# Autodesk Inventor assembly: Granny Gearbox Output Plate Routing Template (8-sheet)
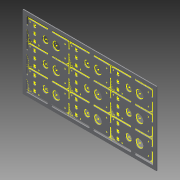
[picture p0: Inventor's stored thumbnail of the model, 180x180]
Saved by Autodesk Inventor 2015 (Build 190159000, 159)
## iProperties
Created: 2016-02-25
Part Number: Granny Gearbox Output Plate Routing Template (8-sheet)
Document SubType Name: Assembly
Designer: sethbattis
Author: sethbattis
## Documents named in this file (4)
- \\area51\team3566\cad\FRC 2016\Granny Gearbox Output Plate Routing Template (8-sheet).iam
- \\area51\team3566\cad\FRC 2016\Granny Gearbox Output Plate Routing Template (border tabs).ipt
- \\area51\team3566\cad\FRC 2016\Granny Gearbox Routing Template Horizontal Tabs.ipt
- \\area51\team3566\cad\FRC 2016\Granny Gearbox Routing Template Vertical Tabs.ipt
## Components (21 placed, 3 different names)
1. Granny Gearbox Output Plate Routing Template (border tabs):1 — Rigid:3, Rigid:4, Rigid:14, Rigid:18
2. Granny Gearbox Output Plate Routing Template (border tabs):2 — Rigid:1, Rigid:2, Rigid:3, Rigid:13
3. Granny Gearbox Output Plate Routing Template (border tabs):3 — Rigid:2, Rigid:7
4. Granny Gearbox Output Plate Routing Template (border tabs):4 — Rigid:6, Rigid:8, Rigid:10
5. Granny Gearbox Output Plate Routing Template (border tabs):5 — Rigid:5, Rigid:6, Rigid:11, Rigid:20
6. Granny Gearbox Output Plate Routing Template (border tabs):6 — Rigid:4, Rigid:5, Rigid:19
7. Granny Gearbox Output Plate Routing Template (border tabs):7 — Rigid:8, Rigid:9, Rigid:17
8. Granny Gearbox Output Plate Routing Template (border tabs):8 — Rigid:7, Rigid:16
9. Granny Gearbox Output Plate Routing Template (border tabs):9 — Rigid:1, Rigid:12, Rigid:15
10. Granny Gearbox Routing Template Horizontal Tabs:1 — Rigid:9
11. Granny Gearbox Routing Template Horizontal Tabs:2 — Rigid:10
12. Granny Gearbox Routing Template Horizontal Tabs:3 — Rigid:11
13. Granny Gearbox Routing Template Horizontal Tabs:4 — Rigid:12
14. Granny Gearbox Routing Template Horizontal Tabs:5 — Rigid:13
15. Granny Gearbox Routing Template Horizontal Tabs:6 — Rigid:14
16. Granny Gearbox Routing Template Vertical Tabs:1 — Rigid:15
17. Granny Gearbox Routing Template Vertical Tabs:2 — Rigid:16
18. Granny Gearbox Routing Template Vertical Tabs:3 — Rigid:17
19. Granny Gearbox Routing Template Vertical Tabs:4 — Rigid:18
20. Granny Gearbox Routing Template Vertical Tabs:5 — Rigid:19
21. Granny Gearbox Routing Template Vertical Tabs:6 — Rigid:20
## Relationships (20: WeldJoint 20)
- Rigid:1 [WeldJoint]: Granny Gearbox Output Plate Routing Template (border tabs):2 ↔ Granny Gearbox Output Plate Routing Template (border tabs):9
- Rigid:2 [WeldJoint]: Granny Gearbox Output Plate Routing Template (border tabs):2 ↔ Granny Gearbox Output Plate Routing Template (border tabs):3
- Rigid:3 [WeldJoint]: Granny Gearbox Output Plate Routing Template (border tabs):1 ↔ Granny Gearbox Output Plate Routing Template (border tabs):2
- Rigid:4 [WeldJoint]: Granny Gearbox Output Plate Routing Template (border tabs):1 ↔ Granny Gearbox Output Plate Routing Template (border tabs):6
- Rigid:5 [WeldJoint]: Granny Gearbox Output Plate Routing Template (border tabs):5 ↔ Granny Gearbox Output Plate Routing Template (border tabs):6
- Rigid:6 [WeldJoint]: Granny Gearbox Output Plate Routing Template (border tabs):4 ↔ Granny Gearbox Output Plate Routing Template (border tabs):5
- Rigid:7 [WeldJoint]: Granny Gearbox Output Plate Routing Template (border tabs):3 ↔ Granny Gearbox Output Plate Routing Template (border tabs):8
- Rigid:8 [WeldJoint]: Granny Gearbox Output Plate Routing Template (border tabs):4 ↔ Granny Gearbox Output Plate Routing Template (border tabs):7
- Rigid:9 [WeldJoint]: Granny Gearbox Output Plate Routing Template (border tabs):7 ↔ Granny Gearbox Routing Template Horizontal Tabs:1
- Rigid:10 [WeldJoint]: Granny Gearbox Output Plate Routing Template (border tabs):4 ↔ Granny Gearbox Routing Template Horizontal Tabs:2
- Rigid:11 [WeldJoint]: Granny Gearbox Output Plate Routing Template (border tabs):5 ↔ Granny Gearbox Routing Template Horizontal Tabs:3
- Rigid:12 [WeldJoint]: Granny Gearbox Output Plate Routing Template (border tabs):9 ↔ Granny Gearbox Routing Template Horizontal Tabs:4
- Rigid:13 [WeldJoint]: Granny Gearbox Output Plate Routing Template (border tabs):2 ↔ Granny Gearbox Routing Template Horizontal Tabs:5
- Rigid:14 [WeldJoint]: Granny Gearbox Output Plate Routing Template (border tabs):1 ↔ Granny Gearbox Routing Template Horizontal Tabs:6
- Rigid:15 [WeldJoint]: Granny Gearbox Output Plate Routing Template (border tabs):9 ↔ Granny Gearbox Routing Template Vertical Tabs:1
- Rigid:16 [WeldJoint]: Granny Gearbox Output Plate Routing Template (border tabs):8 ↔ Granny Gearbox Routing Template Vertical Tabs:2
- Rigid:17 [WeldJoint]: Granny Gearbox Output Plate Routing Template (border tabs):7 ↔ Granny Gearbox Routing Template Vertical Tabs:3
- Rigid:18 [WeldJoint]: Granny Gearbox Output Plate Routing Template (border tabs):1 ↔ Granny Gearbox Routing Template Vertical Tabs:4
- Rigid:19 [WeldJoint]: Granny Gearbox Output Plate Routing Template (border tabs):6 ↔ Granny Gearbox Routing Template Vertical Tabs:5
- Rigid:20 [WeldJoint]: Granny Gearbox Output Plate Routing Template (border tabs):5 ↔ Granny Gearbox Routing Template Vertical Tabs:6
